# Autodesk Inventor assembly: ChestDerived
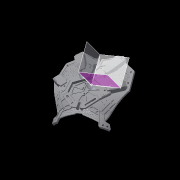
[picture p0: Inventor's stored thumbnail of the model, 180x180]
Saved by Autodesk Inventor 2015 SP1 (Build 190203100, 203)
## iProperties
Created: 2015-05-09
Part Number: ChestDerived
Document SubType Name: Assembly
Designer: Val
Author: Val
## Documents named in this file (5)
- E:\Exo\Models\3D\ChestDerived.iam
- E:\Exo\Models\3D\ChestBaseDerived.ipt
- E:\Exo\Models\3D\ChestPlateRightDerived.ipt
- E:\Exo\Models\3D\ChestPlateLeftDerived.ipt
- E:\Exo\Models\3D\External\Fan12VDC.ipt
## Components (4 placed, 4 different names)
1. ChestBaseDerived:1 — Mate:1, Mate:2, Flush:1, Flush:2
2. ChestPlateRightDerived:1 — Mate:1, Mate:2, Flush:1, Mate:3
3. ChestPlateLeftDerived:1 — Flush:2
4. Fan12VDC:1 — Mate:3
## Relationships (5: Mate 3, Flush 2)
- Mate:1: ChestBaseDerived:1 ↔ ChestPlateRightDerived:1
- Mate:2: ChestBaseDerived:1 ↔ ChestPlateRightDerived:1
- Flush:1: ChestBaseDerived:1 ↔ ChestPlateRightDerived:1
- Flush:2: ChestBaseDerived:1 ↔ ChestPlateLeftDerived:1
- Mate:3: ChestPlateRightDerived:1 ↔ Fan12VDC:1
